# Autodesk Inventor assembly: Knuckle joint
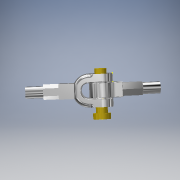
[picture p0: Inventor's stored thumbnail of the model, 180x180]
Saved by Autodesk Inventor 2018 (Build 220112000, 112)
## iProperties
Created: 2019-09-01
Part Number: Knuckle joint
Document SubType Name: Assembly
Designer: Sameer
Author: Sameer
## Documents named in this file (4)
- C:\Users\Sameer\Desktop\Saad\Saad\EMD\Knuckle Joint\Knuckle joint.iam
- C:\Users\Sameer\Desktop\Saad\Saad\EMD\Knuckle Joint\Single Eye End.ipt
- C:\Users\Sameer\Desktop\Saad\Saad\EMD\Knuckle Joint\Double Eye End.ipt
- C:\Users\Sameer\Desktop\Saad\Saad\EMD\Knuckle Joint\Knuckle Pin.ipt
## Components (3 placed, 3 different names)
1. Single Eye End:1 — Mate:1
2. Double Eye End:1 — Mate:1, Mate:2
3. Knuckle Pin:1 — Mate:2
## Relationships (2: Mate 2)
- Mate:1: Single Eye End:1 ↔ Double Eye End:1
- Mate:2: Double Eye End:1 ↔ Knuckle Pin:1
